# Autodesk Inventor assembly: Assembly Ficha de exercícios 4 Exercício 1
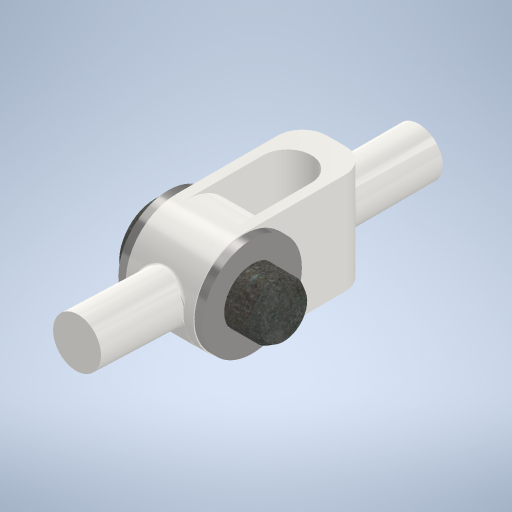
[picture p0: Inventor's stored thumbnail of the model, 512x512]
Saved by Autodesk Inventor 2024 (Build 280153000, 153)
## iProperties
Created: 2024-04-15
Part Number: Assembly Ficha de exercícios 4 Exercício 1
Document SubType Name: Assembly
Designer: Pedro
Author: Pedro
## Documents named in this file (6)
- C:\Users\Pedro\Desktop\Autodesk Inbentor\Aula 7\Assembly Ficha de exercícios 4 Exercício 1.iam
- C:\Users\Pedro\Desktop\Autodesk Inbentor\Aula 7\Forquilha.ipt
- C:\Users\Pedro\Desktop\Autodesk Inbentor\Aula 7\Olhal.ipt
- C:\Users\Pedro\Documents\Inventor\Content Center Files\R2024\en-US\ISO 7089\ISO 7089 - 33 - 140 HV(1).ipt
- C:\Users\Pedro\Documents\Inventor\Content Center Files\R2024\en-US\ISO 2341 B(1)\ISO 2341 - B - 33 x 70ISO.ipt
- C:\Users\Pedro\Documents\Inventor\Content Center Files\R2024\en-US\ISO 2339(2)\ISO 2339 - A - 8 x 35ISO.ipt
## Components (6 placed, 5 different names)
1. Forquilha:1 — Insert:1, Insert:2, Insert:3
2. Olhal:1 — Insert:3
3. ISO 7089 33:1 — Insert:1, Insert:4
4. ISO 7089 33:2 — Insert:2
5. ISO 2341 B B - 33 x 70:1 — Insert:4, Rigid:1
6. ISO 2339 A - 8 x 35:1 — Rigid:1
## Relationships (5: Insert 4, WeldJoint 1)
- Insert:1: Forquilha:1 ↔ ISO 7089 33:1
- Insert:2: Forquilha:1 ↔ ISO 7089 33:2
- Insert:3: Forquilha:1 ↔ Olhal:1
- Insert:4: ISO 7089 33:1 ↔ ISO 2341 B B - 33 x 70:1
- Rigid:1 [WeldJoint]: ISO 2341 B B - 33 x 70:1 ↔ ISO 2339 A - 8 x 35:1
